# Autodesk Inventor assembly: dash_2
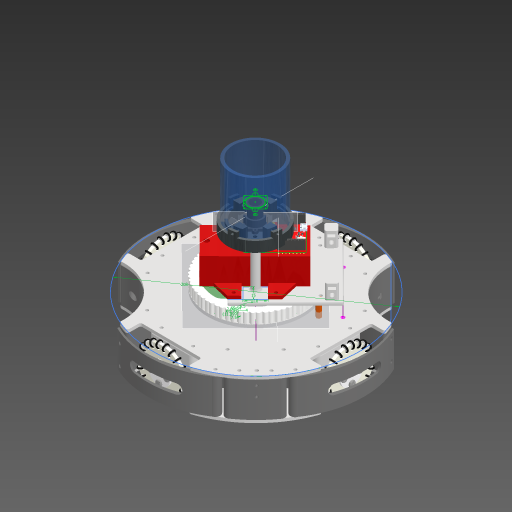
[picture p0: Inventor's stored thumbnail of the model, 512x512]
Saved by Autodesk Inventor 2023 (Build 270158000, 158)
## iProperties
Created: 2025-07-14
Part Number: dash_2
Document SubType Name: Assembly
Designer: daa
Author: daa
## Documents named in this file (8)
- C:\Users\daa\Documents\DASH_V2\dash_2.iam
- C:\Users\daa\Documents\DASH_V2\omni_platforma\omni_platforma.iam
- C:\Users\daa\Documents\DASH_V2\omni_platforma\rack_05.ipt
- C:\Users\daa\Documents\DASH_V2\tssop.iam
- C:\Users\daa\Documents\DASH_V2\Dribler_v2\kreplenie_dribler_V4.ipt
- C:\Users\daa\Documents\DASH_V2\akb_mount.ipt
- C:\Users\daa\Documents\DASH_V2\openmv_cennt.iam
- C:\Users\daa\Documents\DASH_V2\rack_25.ipt
## Components (11 placed, 7 different names)
1. omni_platforma:1 [sub-assembly] — С поворотом:2, С поворотом:3, С поворотом:4, Жесткий:1
2. rack_05:1 — С поворотом:4
3. rack_05:2 — Жесткий:1, С поворотом:11
4. rack_05:3 — С поворотом:2
5. rack_05:4 — С поворотом:3
6. kreplenie_dribler_V4:1 — С поворотом:9, С поворотом:10, Совмещение:1, С поворотом:12
7. akb_mount:1 — С поворотом:9
8. tssop:1 [sub-assembly] — С поворотом:10, Совмещение:1, С поворотом:11
9. openmv_cennt:1 [sub-assembly] — С поворотом:12
10. rack_25:1
11. rack_25:2
## Relationships (9: RevoluteJoint 7, WeldJoint 1, Mate 1)
- С поворотом:2 [RevoluteJoint]: omni_platforma:1 ↔ rack_05:3
- С поворотом:3 [RevoluteJoint]: omni_platforma:1 ↔ rack_05:4
- С поворотом:4 [RevoluteJoint]: omni_platforma:1 ↔ rack_05:1
- Жесткий:1 [WeldJoint]: omni_platforma:1 ↔ rack_05:2
- С поворотом:9 [RevoluteJoint]: kreplenie_dribler_V4:1 ↔ akb_mount:1
- С поворотом:10 [RevoluteJoint]: kreplenie_dribler_V4:1 ↔ tssop:1
- Совмещение:1 [Mate]: kreplenie_dribler_V4:1 ↔ tssop:1
- С поворотом:11 [RevoluteJoint]: rack_05:2 ↔ tssop:1
- С поворотом:12 [RevoluteJoint]: kreplenie_dribler_V4:1 ↔ openmv_cennt:1
